# Autodesk Inventor assembly: ControlHousing
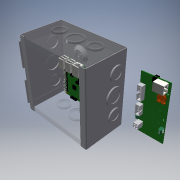
[picture p0: Inventor's stored thumbnail of the model, 180x180]
Saved by Autodesk Inventor 2016 (Build 200138000, 138)
## iProperties
Company: Unknown
Created: 2016-08-11
Part Number: ControlHousing
Description: Unknown
Document SubType Name: Assembly
Designer: jfixelle
Sending System: Unknown
Preprocessor: PSStep 14.0
Title: S:/STOCK/7-COMMERCIAL/CHKO/chko663.stp
Author: Unknown
Revision Number: NONE
## Documents named in this file (16)
- E:\jfixelle\Documents\APC\GitRepo\Control\IAM\ControlHousing.iam
- E:\jfixelle\Downloads\loc13368.ipt
- E:\jfixelle\Downloads\COM55083-4.ipt
- E:\jfixelle\Downloads\COM55563-4.ipt
- E:\jfixelle\Downloads\COM55989.ipt
- E:\jfixelle\Downloads\HNG11000.iam
- E:\jfixelle\Documents\APC\GitRepo\Control\IAM\PiB+.ipt
- E:\jfixelle\Documents\APC\GitRepo\Control\IAM\ControlBoard_New.ipt
- E:\jfixelle\Documents\APC\GitRepo\PCB_Libs\3DParts\IDC_10Pos.ipt
- E:\jfixelle\Documents\APC\GitRepo\PCB_Libs\3DParts\IDC_16Pos.ipt
- E:\jfixelle\Documents\APC\GitRepo\PCB_Libs\3DParts\Molex_MiniFitJR_4Pos.ipt
- E:\jfixelle\Documents\APC\GitRepo\PCB_Libs\3DParts\RJE051AA1310.ipt
- E:\jfixelle\Documents\APC\GitRepo\PCB_Libs\3DParts\H11L1M.ipt
- E:\jfixelle\Documents\APC\GitRepo\PCB_Libs\3DParts\Screw_Terminal_2Pos.ipt
- E:\jfixelle\Documents\APC\GitRepo\PCB_Libs\3DParts\Screw_Terminal_3Pos.ipt
- E:\jfixelle\Documents\APC\GitRepo\PCB_Libs\3DParts\Keystone1056_12_5mmCoinCell.ipt
## Components (18 placed, 17 different names)
1. NAUO4
2. NAUO5
3. NAUO6
4. NAUO7 — Mate:1
5. NAUO8
6. NAUO9 [sub-assembly]
7. NAUO10 [sub-assembly]
8. PiB+:1 — Mate:1
9. ControlBoard_New:1 — Mate:2, Mate:3, Mate:4, Mate:5, Mate:6, Mate:7, Mate:8, Mate:9, Mate:10, Mate:11, Mate:12, Mate:13, Mate:14, Mate:15, Flush:1, Flush:2, Mate:17, Mate:18, Mate:19, Mate:20, Mate:21, Mate:22, Mate:23, Mate:24, Angle:1
10. IDC_10Pos:1 — Mate:2, Mate:7, Mate:8
11. IDC_16Pos:1 — Mate:3, Mate:9, Mate:10
12. Molex_MiniFitJR_4Pos:1 — Mate:4, Mate:5, Mate:6
13. RJE051AA1310:1 — Mate:11, Mate:12, Mate:13, Mate:16
14. H11L1M:1 — Mate:14, Flush:2, Flush:3
15. H11L1M:2 — Mate:15, Flush:1, Mate:16, Flush:3
16. Screw_Terminal_2Pos:1 — Mate:17, Mate:19, Mate:20
17. Screw_Terminal_3Pos:1 — Mate:18, Mate:21, Mate:22
18. Keystone1056_12_5mmCoinCell:1 — Mate:23, Mate:24, Angle:1
## Relationships (28: Mate 24, Flush 3, Angle 1)
- Mate:1 (11 mm): NAUO7 ↔ PiB+:1
- Mate:2: ControlBoard_New:1 ↔ IDC_10Pos:1
- Mate:3: ControlBoard_New:1 ↔ IDC_16Pos:1
- Mate:4: ControlBoard_New:1 ↔ Molex_MiniFitJR_4Pos:1
- Mate:5: ControlBoard_New:1 ↔ Molex_MiniFitJR_4Pos:1
- Mate:6: ControlBoard_New:1 ↔ Molex_MiniFitJR_4Pos:1
- Mate:7: ControlBoard_New:1 ↔ IDC_10Pos:1
- Mate:8: ControlBoard_New:1 ↔ IDC_10Pos:1
- Mate:9: ControlBoard_New:1 ↔ IDC_16Pos:1
- Mate:10: ControlBoard_New:1 ↔ IDC_16Pos:1
- Mate:11: ControlBoard_New:1 ↔ RJE051AA1310:1
- Mate:12: ControlBoard_New:1 ↔ RJE051AA1310:1
- Mate:13: ControlBoard_New:1 ↔ RJE051AA1310:1
- Mate:14: ControlBoard_New:1 ↔ H11L1M:1
- Mate:15: ControlBoard_New:1 ↔ H11L1M:2
- Flush:1: ControlBoard_New:1 ↔ H11L1M:2
- Mate:16: RJE051AA1310:1 ↔ H11L1M:2
- Flush:2: ControlBoard_New:1 ↔ H11L1M:1
- Flush:3: H11L1M:1 ↔ H11L1M:2
- Mate:17: ControlBoard_New:1 ↔ Screw_Terminal_2Pos:1
- Mate:18: ControlBoard_New:1 ↔ Screw_Terminal_3Pos:1
- Mate:19: ControlBoard_New:1 ↔ Screw_Terminal_2Pos:1
- Mate:20: ControlBoard_New:1 ↔ Screw_Terminal_2Pos:1
- Mate:21: ControlBoard_New:1 ↔ Screw_Terminal_3Pos:1
- Mate:22: ControlBoard_New:1 ↔ Screw_Terminal_3Pos:1
- Mate:23: ControlBoard_New:1 ↔ Keystone1056_12_5mmCoinCell:1
- Mate:24: ControlBoard_New:1 ↔ Keystone1056_12_5mmCoinCell:1
- Angle:1 (0 deg): ControlBoard_New:1 ↔ Keystone1056_12_5mmCoinCell:1
